# Autodesk Inventor assembly: ResistojetPrototype
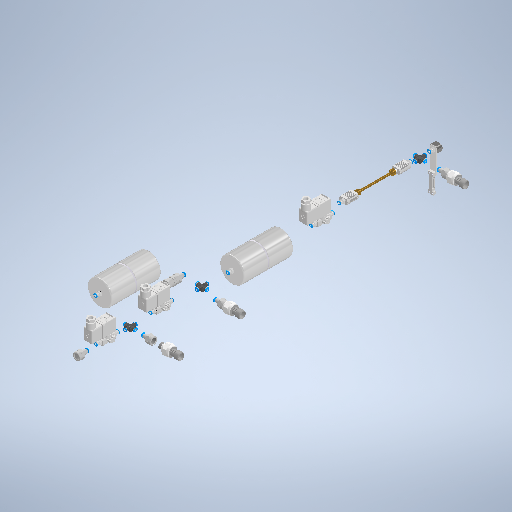
[picture p0: Inventor's stored thumbnail of the model, 512x512]
Saved by Autodesk Inventor 2025.2 (Build 292293000, 293)
## iProperties
Created: 2026-06-11
Part Number: ResistojetPrototype
Document SubType Name: Assembly
Designer: Simon
Author: Simon
## Documents named in this file (17)
- C:\Users\Simon\Projects\MEng Electronics\Development of a Resistojet Thruster\3) Hardware\Resistojet Design\ResistojetV1\ResistojetPrototype.iam
- C:\Users\Simon\Projects\MEng Electronics\Development of a Resistojet Thruster\3) Hardware\Resistojet Design\ResistojetV1\Mechanical Drawings\Heater.ipt
- C:\Users\Simon\Projects\MEng Electronics\Development of a Resistojet Thruster\3) Hardware\Resistojet Design\ResistojetV1\PressureSensor.ipt
- C:\Users\Simon\Projects\MEng Electronics\Development of a Resistojet Thruster\3) Hardware\Resistojet Design\ResistojetV1\Festo_Pneumatic_Coupling_PC4-M10.ipt
- C:\Users\Simon\Projects\MEng Electronics\Development of a Resistojet Thruster\3) Hardware\Resistojet Design\ResistojetV1\Creality Heatsink v1.2.ipt
- C:\Users\Simon\Projects\MEng Electronics\Development of a Resistojet Thruster\3) Hardware\Resistojet Design\ResistojetV1\Heatbreak CR30.ipt
- C:\Users\Simon\Projects\MEng Electronics\Development of a Resistojet Thruster\3) Hardware\Resistojet Design\ResistojetV1\NozzleConnector.ipt
- C:\Users\Simon\Projects\MEng Electronics\Development of a Resistojet Thruster\3) Hardware\Resistojet Design\ResistojetV1\0.4 nozzle.ipt
- C:\Users\Simon\Projects\MEng Electronics\Development of a Resistojet Thruster\3) Hardware\Resistojet Design\ResistojetV1\100g_load_cell.ipt
- C:\Users\Simon\Projects\MEng Electronics\Development of a Resistojet Thruster\3) Hardware\Resistojet Design\ResistojetV1\Loadcell_lever.ipt
- C:\Users\Simon\Projects\MEng Electronics\Development of a Resistojet Thruster\3) Hardware\Resistojet Design\ResistojetV1\ASCO Solenoid Valve\solenoid_valve_scg256a004nvms_4.iam
- C:\Users\Simon\Projects\MEng Electronics\Development of a Resistojet Thruster\3) Hardware\Resistojet Design\ResistojetV1\Mechanical Drawings\WeldedPlenumAssembly.iam
- C:\Users\Simon\Projects\MEng Electronics\Development of a Resistojet Thruster\3) Hardware\Resistojet Design\ResistojetV1\Mechanical Drawings\WeldedTankAssembly.iam
- C:\Users\Simon\Projects\MEng Electronics\Development of a Resistojet Thruster\3) Hardware\Resistojet Design\ResistojetV1\FESTO Parts\153379 QSMX-4.ipt
- C:\Users\Simon\Projects\MEng Electronics\Development of a Resistojet Thruster\3) Hardware\Resistojet Design\ResistojetV1\FESTO Parts\8030272 NPFC-D-2G14-M.ipt
- C:\Users\Simon\Projects\MEng Electronics\Development of a Resistojet Thruster\3) Hardware\Resistojet Design\ResistojetV1\FESTO Parts\8069220 NPFC-R-G14-G18-F.ipt
- C:\Users\Simon\Projects\MEng Electronics\Development of a Resistojet Thruster\3) Hardware\Resistojet Design\ResistojetV1\FESTO Parts\190650 QSF-1_4-4-B.ipt
## Components (39 placed, 16 different names)
1. Heater:1 — Mate:35, Mate:36, Mate:43, Mate:44
2. PressureSensor:2 — Mate:86, Mate:89
3. Festo_Pneumatic_Coupling_PC4-M10:1 — Mate:54, Mate:56
4. Festo_Pneumatic_Coupling_PC4-M10:2 — Mate:47, Mate:48, Mate:49
5. Festo_Pneumatic_Coupling_PC4-M10:3 — Mate:55, Mate:57
6. Festo_Pneumatic_Coupling_PC4-M10:4 — Mate:37, Mate:38
7. Festo_Pneumatic_Coupling_PC4-M10:5 — Mate:74, Mate:75
8. Festo_Pneumatic_Coupling_PC4-M10:6 — Mate:79, Mate:80
9. Creality Heatsink v1.2:1 — Mate:33, Mate:34, Mate:37, Mate:38
10. Heatbreak CR30:1 — Mate:33, Mate:34, Mate:35, Mate:36
11. Festo_Pneumatic_Coupling_PC4-M10:7
12. Creality Heatsink v1.2:2
13. Heatbreak CR30:2 — Mate:43, Mate:44
14. NozzleConnector:1 — Mate:45, Mate:46, Mate:47, Mate:50
15. 0.4 nozzle:1 — Mate:45, Mate:46
16. 100g_load_cell:1 — Mate:51, Mate:52, Mate:53
17. Loadcell_lever:1 — Mate:48, Mate:49, Mate:50, Mate:51, Mate:52, Mate:53
18. solenoid_valve_scg256a004nvms_4:1 [sub-assembly] — Mate:58, Mate:59, Mate:68, Mate:69
19. solenoid_valve_scg256a004nvms_4:2 [sub-assembly] — Mate:54, Mate:55, Mate:56, Mate:57
20. solenoid_valve_scg256a004nvms_4:3 [sub-assembly] — Mate:78, Mate:79, Mate:80, Mate:81
21. Festo_Pneumatic_Coupling_PC4-M10:8 — Mate:59, Mate:68
22. Festo_Pneumatic_Coupling_PC4-M10:9 — Mate:58, Mate:69
23. PressureSensor:4 — Mate:87
24. Festo_Pneumatic_Coupling_PC4-M10:10 — Mate:73, Mate:77
25. Festo_Pneumatic_Coupling_PC4-M10:11 — Mate:72, Mate:76
26. WeldedPlenumAssembly:1 [sub-assembly] — Mate:72, Mate:73, Mate:76, Mate:77
27. WeldedTankAssembly:1 [sub-assembly] — Mate:74, Mate:75
28. Festo_Pneumatic_Coupling_PC4-M10:12 — Mate:78, Mate:81
29. 153379 QSMX-4:1
30. 8030272 NPFC-D-2G14-M:1 — Mate:82, Mate:83, Flush:1, Mate:84, Mate:85
31. 8069220 NPFC-R-G14-G18-F:1 — Mate:84, Mate:85, Flush:2
32. 190650 QSF-1_4-4-B:1 — Mate:82, Mate:83, Flush:1, Flush:2
33. 153379 QSMX-4:2
34. 190650 QSF-1_4-4-B:2 — Mate:88, Mate:90
35. 190650 QSF-1_4-4-B:3 — Mate:87
36. 190650 QSF-1_4-4-B:4
37. 153379 QSMX-4:3
38. PressureSensor:5 — Mate:88, Mate:90
39. 190650 QSF-1_4-4-B:5 — Mate:86, Mate:89
## Relationships (50: Mate 48, Flush 2)
- Mate:33: Creality Heatsink v1.2:1 ↔ Heatbreak CR30:1
- Mate:34: Creality Heatsink v1.2:1 ↔ Heatbreak CR30:1
- Mate:35: Heater:1 ↔ Heatbreak CR30:1
- Mate:36: Heater:1 ↔ Heatbreak CR30:1
- Mate:37: Festo_Pneumatic_Coupling_PC4-M10:4 ↔ Creality Heatsink v1.2:1
- Mate:38: Festo_Pneumatic_Coupling_PC4-M10:4 ↔ Creality Heatsink v1.2:1
- [Mate]: Creality Heatsink v1.2:2 ↔ Heatbreak CR30:2
- [Mate]: Creality Heatsink v1.2:2 ↔ Heatbreak CR30:2
- [Mate]: Festo_Pneumatic_Coupling_PC4-M10:7 ↔ Creality Heatsink v1.2:2
- [Mate]: Festo_Pneumatic_Coupling_PC4-M10:7 ↔ Creality Heatsink v1.2:2
- Mate:43: Heater:1 ↔ Heatbreak CR30:2
- Mate:44: Heater:1 ↔ Heatbreak CR30:2
- Mate:45: NozzleConnector:1 ↔ 0.4 nozzle:1
- Mate:46: NozzleConnector:1 ↔ 0.4 nozzle:1
- Mate:47: Festo_Pneumatic_Coupling_PC4-M10:2 ↔ NozzleConnector:1
- Mate:48: Festo_Pneumatic_Coupling_PC4-M10:2 ↔ Loadcell_lever:1
- Mate:49: Festo_Pneumatic_Coupling_PC4-M10:2 ↔ Loadcell_lever:1
- Mate:50: NozzleConnector:1 ↔ Loadcell_lever:1
- Mate:51: 100g_load_cell:1 ↔ Loadcell_lever:1
- Mate:52: 100g_load_cell:1 ↔ Loadcell_lever:1
- Mate:53: 100g_load_cell:1 ↔ Loadcell_lever:1
- Mate:54: Festo_Pneumatic_Coupling_PC4-M10:1 ↔ solenoid_valve_scg256a004nvms_4:2
- Mate:55: Festo_Pneumatic_Coupling_PC4-M10:3 ↔ solenoid_valve_scg256a004nvms_4:2
- Mate:56: Festo_Pneumatic_Coupling_PC4-M10:1 ↔ solenoid_valve_scg256a004nvms_4:2
- Mate:57: Festo_Pneumatic_Coupling_PC4-M10:3 ↔ solenoid_valve_scg256a004nvms_4:2
- Mate:58: solenoid_valve_scg256a004nvms_4:1 ↔ Festo_Pneumatic_Coupling_PC4-M10:9
- Mate:59: solenoid_valve_scg256a004nvms_4:1 ↔ Festo_Pneumatic_Coupling_PC4-M10:8
- Mate:68: solenoid_valve_scg256a004nvms_4:1 ↔ Festo_Pneumatic_Coupling_PC4-M10:8
- Mate:69: solenoid_valve_scg256a004nvms_4:1 ↔ Festo_Pneumatic_Coupling_PC4-M10:9
- Mate:72: Festo_Pneumatic_Coupling_PC4-M10:11 ↔ WeldedPlenumAssembly:1
- Mate:73: Festo_Pneumatic_Coupling_PC4-M10:10 ↔ WeldedPlenumAssembly:1
- Mate:74: Festo_Pneumatic_Coupling_PC4-M10:5 ↔ WeldedTankAssembly:1
- Mate:75: Festo_Pneumatic_Coupling_PC4-M10:5 ↔ WeldedTankAssembly:1
- Mate:76: Festo_Pneumatic_Coupling_PC4-M10:11 ↔ WeldedPlenumAssembly:1
- Mate:77: Festo_Pneumatic_Coupling_PC4-M10:10 ↔ WeldedPlenumAssembly:1
- Mate:78: solenoid_valve_scg256a004nvms_4:3 ↔ Festo_Pneumatic_Coupling_PC4-M10:12
- Mate:79: Festo_Pneumatic_Coupling_PC4-M10:6 ↔ solenoid_valve_scg256a004nvms_4:3
- Mate:80: Festo_Pneumatic_Coupling_PC4-M10:6 ↔ solenoid_valve_scg256a004nvms_4:3
- Mate:81: solenoid_valve_scg256a004nvms_4:3 ↔ Festo_Pneumatic_Coupling_PC4-M10:12
- Mate:82: 8030272 NPFC-D-2G14-M:1 ↔ 190650 QSF-1_4-4-B:1
- Mate:83: 8030272 NPFC-D-2G14-M:1 ↔ 190650 QSF-1_4-4-B:1
- Flush:1: 8030272 NPFC-D-2G14-M:1 ↔ 190650 QSF-1_4-4-B:1
- Mate:84: 8030272 NPFC-D-2G14-M:1 ↔ 8069220 NPFC-R-G14-G18-F:1
- Mate:85: 8030272 NPFC-D-2G14-M:1 ↔ 8069220 NPFC-R-G14-G18-F:1
- Flush:2: 8069220 NPFC-R-G14-G18-F:1 ↔ 190650 QSF-1_4-4-B:1
- Mate:86: PressureSensor:2 ↔ 190650 QSF-1_4-4-B:5
- Mate:87: PressureSensor:4 ↔ 190650 QSF-1_4-4-B:3
- Mate:88: 190650 QSF-1_4-4-B:2 ↔ PressureSensor:5
- Mate:89: PressureSensor:2 ↔ 190650 QSF-1_4-4-B:5
- Mate:90: 190650 QSF-1_4-4-B:2 ↔ PressureSensor:5
## Named parameters: d43_d37 = 0 mm, d44_d38 = 0 mm, d45_d41 = 0 mm, d46_d42 = 0 mm
